# Autodesk Inventor assembly: Intake 2
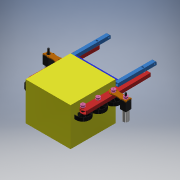
[picture p0: Inventor's stored thumbnail of the model, 180x180]
Saved by Autodesk Inventor 2017 SP1 (Build 210196100, 196)
## iProperties
Created: 2018-01-23
Part Number: Intake 2
Document SubType Name: Assembly
Designer: Ben
Mass: 2492.9 g
Surface Area: 13580.9 cm^2
Volume: 31878.5 cm^3
Density: 0.0782001 g/cm^3
Author: Ben
## Documents named in this file (10)
- C:\Users\Ben\Desktop\Projects\2018 Robot\Cube Intake\Intake 2.iam
- C:\Users\Ben\Desktop\Projects\2018 Robot\Cube Intake\arm.ipt
- C:\Users\Ben\Desktop\Projects\2018 Robot\Cube Intake\intake roller.ipt
- C:\Users\Ben\Desktop\Projects\2018 Robot\Cube Lift\cube.ipt
- C:\Users\Ben\Desktop\Projects\2018 Robot\Cube Intake\pivot arm.ipt
- C:\Users\Ben\Desktop\Projects\2018 Robot\Cube Intake\cross brace.ipt
- C:\Users\Ben\Desktop\Projects\2018 Robot\Cube Intake\rest plate.ipt
- C:\Users\Ben\Desktop\Projects\2018 Robot\Cube Intake\micro cim.ipt
- C:\Users\Ben\Desktop\Projects\2018 Robot\Cube Intake\Part69.ipt
- C:\Users\Ben\Desktop\Projects\2018 Robot\Cube Intake\1277N450_CORROSION-RESISTANT TIMING BELT PULLEY.ipt
## Components (25 placed, 9 different names)
1. arm:1 — Symmetry:1, Insert:1, Insert:2, Insert:3, Insert:10, Insert:15, Insert:16, Mate:17, Mate:18
2. arm:2 — Symmetry:1, Insert:4, Insert:5, Insert:6, Insert:7, Insert:11, Insert:12, Mate:19, Mate:20
3. intake roller:1 — Insert:2
4. intake roller:2 — Insert:1, Tangent:1
5. intake roller:3 — Insert:6
6. intake roller:4 — Insert:4
7. intake roller:5 — Insert:5
8. intake roller:6 — Insert:3
9. cube:1 — Mate:5, Flush:2, Tangent:1
10. pivot arm:1 — Mate:6, Mate:7, Mate:8, Flush:3, Symmetry:2, Insert:7, Mate:16
11. pivot arm:2 — Mate:8, Flush:3, Symmetry:2, Angle:1, Flush:4, Flush:5, Mate:10, Insert:10
12. cross brace:1 — Flush:4, Flush:5, Mate:10, Mate:11, Flush:6, Mate:16
13. rest plate:1 — Mate:11, Flush:6, Flush:7
14. micro cim:1 — Insert:13, Insert:14
15. Part69:1 — Insert:11, Insert:12, Insert:13, Insert:14, Insert:21, Insert:22
16. Part69:2 — Insert:15, Insert:16, Insert:17, Insert:18, Insert:19, Insert:20
17. micro cim:2 — Insert:17, Insert:18
18. 1277N450_CORROSION-RESISTANT TIMING BELT PULLEY:1 — Insert:19
19. 1277N450_CORROSION-RESISTANT TIMING BELT PULLEY:2 — Mate:17, Flush:8
20. 1277N450_CORROSION-RESISTANT TIMING BELT PULLEY:3 — Mate:18, Flush:9
21. 1277N450_CORROSION-RESISTANT TIMING BELT PULLEY:4 — Insert:20, Flush:8, Flush:9
22. 1277N450_CORROSION-RESISTANT TIMING BELT PULLEY:5 — Insert:21
23. 1277N450_CORROSION-RESISTANT TIMING BELT PULLEY:6 — Insert:22, Flush:10, Flush:11
24. 1277N450_CORROSION-RESISTANT TIMING BELT PULLEY:7 — Mate:19, Flush:10
25. 1277N450_CORROSION-RESISTANT TIMING BELT PULLEY:8 — Mate:20, Flush:11
## Relationships (45: Insert 20, Mate 11, Flush 10, Symmetry 2, Angle 1, Tangent 1)
- Symmetry:1: arm:1 ↔ arm:2
- Insert:1 (3.175 mm): arm:1 ↔ intake roller:2
- Insert:2 (3.175 mm): arm:1 ↔ intake roller:1
- Insert:3 (3.175 mm): arm:1 ↔ intake roller:6
- Insert:4 (3.175 mm): arm:2 ↔ intake roller:4
- Insert:5 (3.175 mm): arm:2 ↔ intake roller:5
- Insert:6 (3.175 mm): arm:2 ↔ intake roller:3
- Mate:5 (-247.65 mm): cube:1
- Flush:2: cube:1
- Mate:6: pivot arm:1
- Mate:7: pivot arm:1
- Mate:8: pivot arm:1 ↔ pivot arm:2
- Flush:3: pivot arm:1 ↔ pivot arm:2
- Symmetry:2: pivot arm:1 ↔ pivot arm:2
- Insert:7 (1.5875 mm): arm:2 ↔ pivot arm:1
- Angle:1 (0 deg): pivot arm:2
- Tangent:1 (25.4 mm): intake roller:2 ↔ cube:1
- Flush:4: pivot arm:2 ↔ cross brace:1
- Flush:5: pivot arm:2 ↔ cross brace:1
- Mate:10: pivot arm:2 ↔ cross brace:1
- Mate:11: cross brace:1 ↔ rest plate:1
- Flush:6: cross brace:1 ↔ rest plate:1
- Flush:7: rest plate:1
- Mate:16: pivot arm:1 ↔ cross brace:1
- Insert:10 (1.5875 mm): arm:1 ↔ pivot arm:2
- Insert:11: arm:2 ↔ Part69:1
- Insert:12: arm:2 ↔ Part69:1
- Insert:13: micro cim:1 ↔ Part69:1
- Insert:14: micro cim:1 ↔ Part69:1
- Insert:15: arm:1 ↔ Part69:2
- Insert:16: arm:1 ↔ Part69:2
- Insert:17: Part69:2 ↔ micro cim:2
- Insert:18: Part69:2 ↔ micro cim:2
- Insert:19 (1.5875 mm): Part69:2 ↔ 1277N450_CORROSION-RESISTANT TIMING BELT PULLEY:1
- Insert:20 (1.5875 mm): Part69:2 ↔ 1277N450_CORROSION-RESISTANT TIMING BELT PULLEY:4
- Mate:17: arm:1 ↔ 1277N450_CORROSION-RESISTANT TIMING BELT PULLEY:2
- Mate:18: arm:1 ↔ 1277N450_CORROSION-RESISTANT TIMING BELT PULLEY:3
- Flush:8: 1277N450_CORROSION-RESISTANT TIMING BELT PULLEY:2 ↔ 1277N450_CORROSION-RESISTANT TIMING BELT PULLEY:4
- Flush:9: 1277N450_CORROSION-RESISTANT TIMING BELT PULLEY:3 ↔ 1277N450_CORROSION-RESISTANT TIMING BELT PULLEY:4
- Insert:21 (1.5875 mm): Part69:1 ↔ 1277N450_CORROSION-RESISTANT TIMING BELT PULLEY:5
- Insert:22 (1.5875 mm): Part69:1 ↔ 1277N450_CORROSION-RESISTANT TIMING BELT PULLEY:6
- Mate:19: arm:2 ↔ 1277N450_CORROSION-RESISTANT TIMING BELT PULLEY:7
- Mate:20: arm:2 ↔ 1277N450_CORROSION-RESISTANT TIMING BELT PULLEY:8
- Flush:10: 1277N450_CORROSION-RESISTANT TIMING BELT PULLEY:6 ↔ 1277N450_CORROSION-RESISTANT TIMING BELT PULLEY:7
- Flush:11: 1277N450_CORROSION-RESISTANT TIMING BELT PULLEY:6 ↔ 1277N450_CORROSION-RESISTANT TIMING BELT PULLEY:8
